# Autodesk Inventor assembly: Mechunam base 1.10
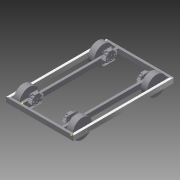
[picture p0: Inventor's stored thumbnail of the model, 180x180]
Saved by Autodesk Inventor 2015 (Build 190159000, 159)
## iProperties
Created: 2015-01-11
Part Number: Mechunam base 1.10
Document SubType Name: Weldment
Designer: chapale16
Weld Material: Welded Aluminum-6061
Author: chapale16
## Documents named in this file (9)
- H:\Mechunam base 1.10.iam
- H:\42in 2x1 boxbeam.ipt
- H:\40in 2x1 boxbeam.ipt
- H:\28in 1x2.ipt
- H:\40in 2x1 boxbeam_MIR_MIR.ipt
- H:\28in 1x2_MIR1_MIR.ipt
- H:\42in 2x1 boxbeam_MIR1_MIR.ipt
- H:\Toughbox-mini.iam
- H:\Mechanum.ipt
## Components (14 placed, 8 different names)
1. 40in 2x1 boxbeam:4 — Mate:3, Mate:4, Mate:24, Mate:26
2. 28in 1x2:1 — Mate:1, Mate:2, Mate:4
3. 42in 2x1 boxbeam:2 — Mate:1, Mate:2, Mate:3, Mate:17, Mate:18, Mate:19, Mate:20, Mate:21
4. 40in 2x1 boxbeam_MIR_MIR:1 — Mate:13, Mate:14, Mate:22, Mate:23, Mate:25, Mate:27
5. 28in 1x2_MIR1_MIR:1 — Mate:13, Mate:15, Mate:16, Mate:17, Mate:18
6. 42in 2x1 boxbeam_MIR1_MIR:1 — Mate:14, Mate:15, Mate:16
7. Mechanum:1 — Mate:19, Mate:21
8. Mechanum:2 — Mate:20
9. Mechanum:3 — Mate:22
10. Mechanum:4 — Mate:23
11. Toughbox-mini:1 [sub-assembly] — Mate:27
12. Toughbox-mini:2 [sub-assembly] — Mate:25
13. Toughbox-mini:3 [sub-assembly] — Mate:26
14. Toughbox-mini:4 [sub-assembly] — Mate:24
## Relationships (19: Mate 19)
- Mate:1: 28in 1x2:1 ↔ 42in 2x1 boxbeam:2
- Mate:2: 28in 1x2:1 ↔ 42in 2x1 boxbeam:2
- Mate:3 (98.425 mm): 40in 2x1 boxbeam:4 ↔ 42in 2x1 boxbeam:2
- Mate:4: 40in 2x1 boxbeam:4 ↔ 28in 1x2:1
- Mate:13: 40in 2x1 boxbeam_MIR_MIR:1 ↔ 28in 1x2_MIR1_MIR:1
- Mate:14 (98.425 mm): 40in 2x1 boxbeam_MIR_MIR:1 ↔ 42in 2x1 boxbeam_MIR1_MIR:1
- Mate:15: 28in 1x2_MIR1_MIR:1 ↔ 42in 2x1 boxbeam_MIR1_MIR:1
- Mate:16: 28in 1x2_MIR1_MIR:1 ↔ 42in 2x1 boxbeam_MIR1_MIR:1
- Mate:17: 42in 2x1 boxbeam:2 ↔ 28in 1x2_MIR1_MIR:1
- Mate:18: 42in 2x1 boxbeam:2 ↔ 28in 1x2_MIR1_MIR:1
- Mate:19 (17.145 mm): 42in 2x1 boxbeam:2 ↔ Mechanum:1
- Mate:20 (42.545 mm): 42in 2x1 boxbeam:2 ↔ Mechanum:2
- Mate:21 (42.545 mm): 42in 2x1 boxbeam:2 ↔ Mechanum:1
- Mate:22 (42.545 mm): 40in 2x1 boxbeam_MIR_MIR:1 ↔ Mechanum:3
- Mate:23 (42.545 mm): 40in 2x1 boxbeam_MIR_MIR:1 ↔ Mechanum:4
- Mate:24: 40in 2x1 boxbeam:4 ↔ Toughbox-mini:4
- Mate:25: 40in 2x1 boxbeam_MIR_MIR:1 ↔ Toughbox-mini:2
- Mate:26: 40in 2x1 boxbeam:4 ↔ Toughbox-mini:3
- Mate:27: 40in 2x1 boxbeam_MIR_MIR:1 ↔ Toughbox-mini:1
